# Autodesk Inventor assembly: ASY ДМФ 0110 крышка галка
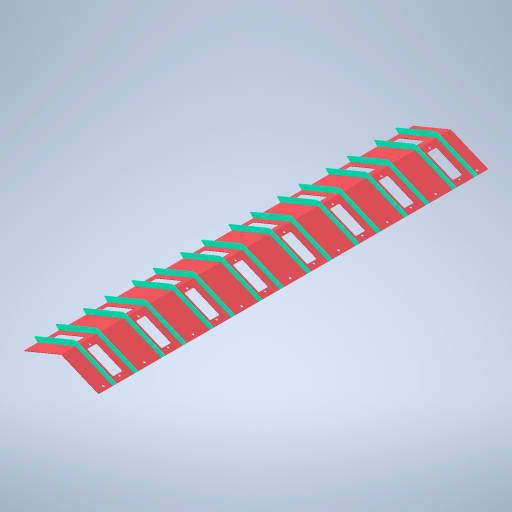
[picture p0: Inventor's stored thumbnail of the model, 512x512]
Saved by Autodesk Inventor 2024.2 (Build 282272000, 272)
## iProperties
Created: 2024-04-30
Part Number: ASY ДМФ 0110 крышка галка
Document SubType Name: Assembly
Designer: admin
Author: admin
## Documents named in this file (3)
- C:\Users\admin\Documents\Inventor\DMF-Disk-Micro-Filter\ASY ДМФ 0110 крышка галка.iam
- C:\Users\admin\Documents\Inventor\DMF-Disk-Micro-Filter\ДМФ 0111 Барабан Лист крышка.ipt
- C:\Users\admin\Documents\Inventor\DMF-Disk-Micro-Filter\ДМФ 0112 Сектор кольца усилителя барабана_CPY.ipt
## Components (17 placed, 2 different names)
1. ДМС 100 Барабан Лист №1:1 — Mate:1, Mate:2, Flush:1
2. ДМС 104 Сектор кольца усилителя барабана_CPY:2 — Rigid:1
3. ДМС 104 Сектор кольца усилителя барабана_CPY:1 — Mate:1, Mate:2, Rigid:1
4. ДМС 104 Сектор кольца усилителя барабана_CPY:3
5. ДМС 104 Сектор кольца усилителя барабана_CPY:4
6. ДМС 104 Сектор кольца усилителя барабана_CPY:5
7. ДМС 104 Сектор кольца усилителя барабана_CPY:6
8. ДМС 104 Сектор кольца усилителя барабана_CPY:7
9. ДМС 104 Сектор кольца усилителя барабана_CPY:8
10. ДМС 104 Сектор кольца усилителя барабана_CPY:9
11. ДМС 104 Сектор кольца усилителя барабана_CPY:10
12. ДМС 104 Сектор кольца усилителя барабана_CPY:11
13. ДМС 104 Сектор кольца усилителя барабана_CPY:12
14. ДМС 104 Сектор кольца усилителя барабана_CPY:13
15. ДМС 104 Сектор кольца усилителя барабана_CPY:14
16. ДМС 104 Сектор кольца усилителя барабана_CPY:15 — Flush:1
17. ДМС 104 Сектор кольца усилителя барабана_CPY:16
## Component patterns: (8 elements, first: ДМС 104 Сектор кольца усилителя барабана_CPY:2 + ДМС 104 Сектор кольца усилителя барабана_CPY:1)
## Relationships (4: Mate 2, WeldJoint 1, Flush 1)
- Mate:1: ДМС 100 Барабан Лист №1:1 ↔ ДМС 104 Сектор кольца усилителя барабана_CPY:1
- Mate:2: ДМС 100 Барабан Лист №1:1 ↔ ДМС 104 Сектор кольца усилителя барабана_CPY:1
- Rigid:1 [WeldJoint] (108 mm): ДМС 104 Сектор кольца усилителя барабана_CPY:2 ↔ ДМС 104 Сектор кольца усилителя барабана_CPY:1
- Flush:1 (29 mm): ДМС 100 Барабан Лист №1:1 ↔ ДМС 104 Сектор кольца усилителя барабана_CPY:15
